# Autodesk Inventor assembly: Assembly3
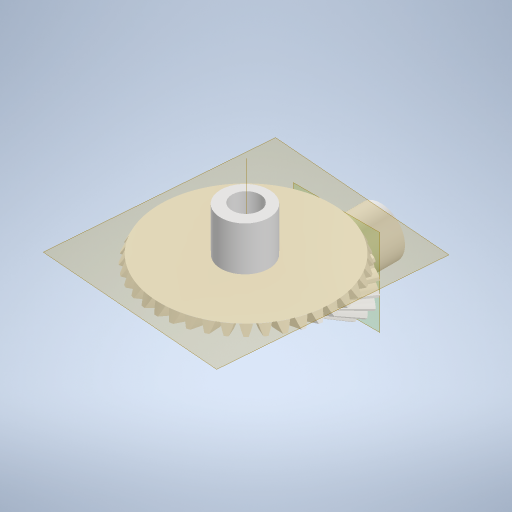
[picture p0: Inventor's stored thumbnail of the model, 512x512]
Saved by Autodesk Inventor 2024 (Build 280153000, 153)
## iProperties
Created: 2023-08-25
Part Number: Assembly3
Document SubType Name: Assembly
Designer: katch
Author: katch
## Documents named in this file (3)
- C:\Users\katch\OneDrive\Documents\TA201&TA202\Assembly3.iam
- C:\Users\katch\OneDrive\Documents\TA201&TA202\Assembly3\Design Accelerator\Bevel Gears1.iam
- C:\Users\katch\OneDrive\Documents\TA201&TA202\Part7.ipt
## Components (2 placed, 2 different names)
1. Bevel Gears:1 [sub-assembly] — Flush:1, Flush:2, Flush:3
2. Part7:1 — Flush:1, Flush:2, Flush:3
## Relationships (3: Flush 3)
- Flush:1: Bevel Gears:1 ↔ Part7:1
- Flush:2: Bevel Gears:1 ↔ Part7:1
- Flush:3: Bevel Gears:1 ↔ Part7:1
